# Autodesk Inventor assembly: MotorMountAssembly2021-Nov
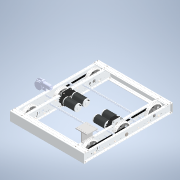
[picture p0: Inventor's stored thumbnail of the model, 180x180]
Saved by Autodesk Inventor 2022.1 (Build 261234020, 234B)
## iProperties
Created: 2021-11-10
Part Number: MotorMountAssembly2021-Nov
Document SubType Name: Assembly
Designer: robst
Author: robst
## Documents named in this file (5)
- C:\git\CAD-Development\robSteele\MotorMountAssembly2021-Nov.iam
- C:\git\CAD-MfgResources\Andy-Mark\MotorMounts\am-2373 Snow Blower Motor Mount.ipt
- C:\git\CAD-MfgResources\Andy-Mark\Motors\SnowBlowerMotor\AM-2235.iam
- C:\git\CAD-Development\robSteele\2020LongRobotBase\AM14U4 Long.iam
- C:\git\CAD-Development\robSteele\pullyBracket.ipt
## Components (4 placed, 4 different names)
1. am-2373 Snow Blower Motor Mount:1 — Insert:2, Insert:3
2. AM-2235:1 [sub-assembly] — Insert:2, Insert:3
3. AM14U4 Long:1 [sub-assembly] — Insert:4, Insert:5
4. pullyBracket:1 — Insert:4, Insert:5
## Relationships (4: Insert 4)
- Insert:2: am-2373 Snow Blower Motor Mount:1 ↔ AM-2235:1
- Insert:3: am-2373 Snow Blower Motor Mount:1 ↔ AM-2235:1
- Insert:4: AM14U4 Long:1 ↔ pullyBracket:1
- Insert:5: AM14U4 Long:1 ↔ pullyBracket:1
